# Autodesk Inventor assembly: Assembly_BREAD
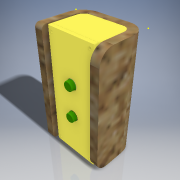
[picture p0: Inventor's stored thumbnail of the model, 180x180]
Saved by Autodesk Inventor 2017 (Build 210142000, 142)
## iProperties
Created: 2019-09-14
Part Number: Assembly_BREAD
Document SubType Name: Assembly
Designer: Admin
Author: Admin
## Documents named in this file (7)
- C:\NTU\DIP\dip 3d sketch\ICE CREAM\Assembly_BREAD.iam
- C:\NTU\DIP\dip 3d sketch\ICE CREAM\BREAD.ipt
- C:\NTU\DIP\dip 3d sketch\ICE CREAM\ICE CREAM COVER.ipt
- C:\NTU\DIP\dip 3d sketch\ICE CREAM\ICE CREAM.ipt
- C:\NTU\DIP\dip 3d sketch\ICE CREAM\BTN_2.ipt
- C:\NTU\DIP\dip 3d sketch\ICE CREAM\BTN_1.ipt
- C:\NTU\DIP\dip 3d sketch\ICE CREAM\BTN_3.ipt
## Components (9 placed, 6 different names)
1. BREAD:1 — Mate:1, Mate:2, Mate:3
2. ICE CREAM COVER:1 — Mate:4, Mate:5, Mate:6, Mate:17, Insert:1, Mate:24, Insert:2
3. ICE CREAM:1 — Mate:1, Mate:2, Mate:3, Mate:4, Mate:5, Mate:6
4. BTN_2:1 — Mate:7, Mate:8, Mate:9, Mate:10, Mate:11, Mate:12, Mate:13, Mate:14, Mate:15, Mate:16
5. BTN_1:1 — Mate:7, Mate:8, Mate:9
6. BTN_3:1 — Mate:10, Mate:11, Mate:12, Mate:13, Mate:14, Mate:15, Mate:16, Mate:17, Insert:1
7. BTN_3:2 — Mate:21, Mate:22, Mate:23, Mate:24, Insert:2
8. BTN_2:2 — Mate:18, Mate:19, Mate:20, Mate:21, Mate:22, Mate:23
9. BTN_1:2 — Mate:18, Mate:19, Mate:20
## Relationships (26: Mate 24, Insert 2)
- Mate:1: BREAD:1 ↔ ICE CREAM:1
- Mate:2: BREAD:1 ↔ ICE CREAM:1
- Mate:3: BREAD:1 ↔ ICE CREAM:1
- Mate:4: ICE CREAM COVER:1 ↔ ICE CREAM:1
- Mate:5: ICE CREAM COVER:1 ↔ ICE CREAM:1
- Mate:6: ICE CREAM COVER:1 ↔ ICE CREAM:1
- Mate:7: BTN_2:1 ↔ BTN_1:1
- Mate:8: BTN_2:1 ↔ BTN_1:1
- Mate:9: BTN_2:1 ↔ BTN_1:1
- Mate:10: BTN_2:1 ↔ BTN_3:1
- Mate:11: BTN_2:1 ↔ BTN_3:1
- Mate:12: BTN_2:1 ↔ BTN_3:1
- Mate:13: BTN_2:1 ↔ BTN_3:1
- Mate:14: BTN_2:1 ↔ BTN_3:1
- Mate:15: BTN_2:1 ↔ BTN_3:1
- Mate:16: BTN_2:1 ↔ BTN_3:1
- Mate:17: ICE CREAM COVER:1 ↔ BTN_3:1
- Insert:1: ICE CREAM COVER:1 ↔ BTN_3:1
- Mate:18: BTN_2:2 ↔ BTN_1:2
- Mate:19: BTN_2:2 ↔ BTN_1:2
- Mate:20: BTN_2:2 ↔ BTN_1:2
- Mate:21: BTN_3:2 ↔ BTN_2:2
- Mate:22: BTN_3:2 ↔ BTN_2:2
- Mate:23: BTN_3:2 ↔ BTN_2:2
- Mate:24: ICE CREAM COVER:1 ↔ BTN_3:2
- Insert:2: ICE CREAM COVER:1 ↔ BTN_3:2
